# Autodesk Inventor assembly: 4th 5th and 6th Axes Model Assembly
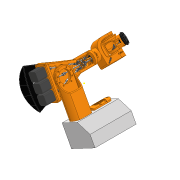
[picture p0: Inventor's stored thumbnail of the model, 180x180]
Saved by Autodesk Inventor 2020 (Build 240168000, 168)
## iProperties
Created: 2021-06-26
Part Number: 4th 5th and 6th Axes Model Assembly
Document SubType Name: Assembly
Designer: Coy
Author: Coy
## Documents named in this file (39)
- E:\Documents\3D Files\Project 3D Models\Industrial 6 Axis Robot Arm\4th 5th amd 6th axis model\4th 5th and 6th Axes Model Assembly.iam
- E:\Documents\3D Files\Project 3D Models\Industrial 6 Axis Robot Arm\4th 5th amd 6th axis model\4th Axis Barrel.ipt
- E:\Documents\3D Files\Project 3D Models\Industrial 6 Axis Robot Arm\4th 5th amd 6th axis model\40mm Bearing.ipt
- E:\Documents\3D Files\Project 3D Models\Industrial 6 Axis Robot Arm\4th 5th amd 6th axis model\5th Axis Tube.ipt
- E:\Documents\3D Files\Project 3D Models\Industrial 6 Axis Robot Arm\4th 5th amd 6th axis model\5x100mm Rod.ipt
- E:\Documents\3D Files\Project 3D Models\Industrial 6 Axis Robot Arm\4th 5th amd 6th axis model\3rd Axis.ipt
- E:\Documents\3D Files\Project 3D Models\Industrial 6 Axis Robot Arm\4th 5th amd 6th axis model\5x8x2.5mm Bearing.ipt
- E:\Documents\3D Files\Project 3D Models\Industrial 6 Axis Robot Arm\4th 5th amd 6th axis model\12x28x8mm Bearing.ipt
- E:\Documents\3D Files\Project 3D Models\Industrial 6 Axis Robot Arm\4th 5th amd 6th axis model\4th Axis Drive Gears.ipt
- E:\Documents\3D Files\Project 3D Models\Industrial 6 Axis Robot Arm\4th 5th amd 6th axis model\6th Axis Drive Gear.ipt
- E:\Documents\3D Files\Project 3D Models\Industrial 6 Axis Robot Arm\4th 5th amd 6th axis model\5x60mm Rod.ipt
- E:\Documents\3D Files\Project 3D Models\Industrial 6 Axis Robot Arm\4th 5th amd 6th axis model\4th Axis Main Drive Gear.ipt
- E:\Documents\3D Files\Project 3D Models\Industrial 6 Axis Robot Arm\4th 5th amd 6th axis model\5th Axis Drive Gear.ipt
- E:\Documents\3D Files\Project 3D Models\Industrial 6 Axis Robot Arm\4th 5th amd 6th axis model\5x42mm Rod.ipt
- E:\Documents\3D Files\Project 3D Models\Industrial 6 Axis Robot Arm\4th 5th amd 6th axis model\5x31mm Rod.ipt
- E:\Documents\3D Files\Project 3D Models\Industrial 6 Axis Robot Arm\4th 5th amd 6th axis model\5x24mm Universal Joint\Assembly.iam
- E:\Documents\3D Files\Project 3D Models\Industrial 6 Axis Robot Arm\4th 5th amd 6th axis model\Nema 17 Stepper Motor.ipt
- E:\Documents\3D Files\Project 3D Models\Industrial 6 Axis Robot Arm\4th 5th amd 6th axis model\5x61.5mm Rod.ipt
- E:\Documents\3D Files\Project 3D Models\Industrial 6 Axis Robot Arm\4th 5th amd 6th axis model\5mm Coupler.ipt
- E:\Documents\3D Files\Project 3D Models\Industrial 6 Axis Robot Arm\4th 5th amd 6th axis model\5x67.3mm Rod.ipt
- E:\Documents\3D Files\Downloaded 3D Files\GrabCad Downloads\gt2-belt-timing-gears-1.snapshot.15\STEP\Gear-5mm-36teeth.ipt
- E:\Documents\3D Files\Downloaded 3D Files\GrabCad Downloads\gt2-belt-timing-gears-1.snapshot.15\STEP\Gear-10mm-36teeth.ipt
- E:\Documents\3D Files\Project 3D Models\Industrial 6 Axis Robot Arm\4th 5th amd 6th axis model\GT2 Idler Pulley.ipt
- E:\Documents\3D Files\Project 3D Models\Industrial 6 Axis Robot Arm\4th 5th amd 6th axis model\M5 60mm Threaded Rod.ipt
- E:\Documents\3D Files\Project 3D Models\Industrial 6 Axis Robot Arm\4th 5th amd 6th axis model\Axis 6 Gearbox.ipt
- E:\Documents\3D Files\Project 3D Models\Industrial 6 Axis Robot Arm\4th 5th amd 6th axis model\Axis 5 Drive Rod.ipt
- E:\Documents\3D Files\Project 3D Models\Industrial 6 Axis Robot Arm\4th 5th amd 6th axis model\Mounting Plate.ipt
- E:\Documents\3D Files\Project 3D Models\Industrial 6 Axis Robot Arm\4th 5th amd 6th axis model\25x37x7mm Bearing.ipt
- E:\Documents\3D Files\Project 3D Models\Industrial 6 Axis Robot Arm\4th 5th amd 6th axis model\5x37.5mm Rod.ipt
- E:\Documents\3D Files\Project 3D Models\Industrial 6 Axis Robot Arm\4th 5th amd 6th axis model\5x45.75mm Rod.ipt
- E:\Documents\3D Files\Project 3D Models\Industrial 6 Axis Robot Arm\4th 5th amd 6th axis model\Corner Gear.ipt
- E:\Documents\3D Files\Project 3D Models\Industrial 6 Axis Robot Arm\4th 5th amd 6th axis model\5th Axis Cover.ipt
- E:\Documents\3D Files\Project 3D Models\Industrial 6 Axis Robot Arm\4th 5th amd 6th axis model\Motor Gard.ipt
- E:\Documents\3D Files\Project 3D Models\Industrial 6 Axis Robot Arm\4th 5th amd 6th axis model\Axis 2 Arm.ipt
- E:\Documents\3D Files\Project 3D Models\Industrial 6 Axis Robot Arm\4th 5th amd 6th axis model\Axis 6 Gearbox Bearing Attchment.ipt
- E:\Documents\3D Files\Project 3D Models\Industrial 6 Axis Robot Arm\4th 5th amd 6th axis model\KR500 0.25 Model Stand.ipt
- E:\Documents\3D Files\Project 3D Models\Industrial 6 Axis Robot Arm\4th 5th amd 6th axis model\3rd Axis Motor Mounts.ipt
- E:\Documents\3D Files\Project 3D Models\Industrial 6 Axis Robot Arm\4th 5th amd 6th axis model\GT2 Idler Pulley No Walls.ipt
- C:\Users\Coy\Downloads\2664N316_METAL GEAR - 20 DEGREE PRESSURE ANGLE.ipt
## Components (80 placed, 38 different names)
1. 4th Axis Barrel:1 — Mate:1, Mate:2, Mate:14, Flush:4, Mate:21, Rotation:2, Rotation:3, Flush:33, Mate:71, Flush:34, Flush:35, Flush:38, Flush:39, Mate:107, Flush:51, Mate:108, Mate:119, Mate:128
2. 40mm Bearing:1 — Mate:1, Mate:2, Mate:10
3. 5th Axis Tube:1 — Flush:1, Flush:2, Mate:13, Mate:16, Flush:3, Flush:4, Flush:21, Flush:22, Rotation:14, Flush:36, Rotation:29
4. 5x100mm Rod:1 — Mate:11, Mate:12, Mate:15, Mate:16, Flush:3, Mate:22, Flush:10, Rotation:4, Mate:27, Flush:37, Rotation:30
5. 3rd Axis:1 — Mate:10, Mate:15, Mate:17, Mate:18, Flush:7, Flush:8, Mate:21, Mate:28, Flush:14, Mate:29, Flush:15, Mate:30, Flush:16, Mate:31, Flush:17, Mate:32, Flush:18, Mate:40, Flush:25, Mate:41, Flush:26, Angle:1, Angle:2, Angle:3, Mate:110, Mate:111, Mate:112, Mate:113, Mate:114, Mate:122, Mate:123, Mate:124
6. 5x8x2.5mm Bearing:1 — Mate:11, Flush:1
7. 5x8x2.5mm Bearing:2 — Mate:12, Flush:2
8. 12x28x8mm Bearing:1 — Mate:13, Mate:14
9. 4th Axis Drive Gears:1 — Mate:20, Rotation:3, Flush:12
10. 4th Axis Drive Gears:2 — Mate:19, Rotation:2, Flush:11
11. 5x8x2.5mm Bearing:3 — Mate:17, Flush:7, Mate:19, Mate:23
12. 5x8x2.5mm Bearing:4 — Mate:18, Flush:8, Mate:20, Mate:24
13. 6th Axis Drive Gear:1 — Mate:22, Flush:10, Rotation:4, Flush:23, Flush:24, Rotation:15
14. 5x60mm Rod:1 — Mate:23, Flush:11, Rotation:10
15. 5x60mm Rod:2 — Mate:24, Flush:12, Mate:34, Rotation:8
16. 5x100mm Rod:2 — Mate:25, Flush:13, Mate:27, Mate:33, Mate:64, Mate:65, Mate:67, Rotation:27
17. 4th Axis Drive Gears:3 — Mate:25, Flush:13, Flush:19, Rotation:9, Flush:20
18. 4th Axis Main Drive Gear:1 — Mate:34, Flush:19, Rotation:8, Rotation:9
19. 4th Axis Main Drive Gear:2 — Flush:20, Rotation:10
20. 5x8x2.5mm Bearing:5 — Mate:28, Flush:14
21. 5x8x2.5mm Bearing:6 — Mate:31, Flush:17, Mate:33
22. 5x8x2.5mm Bearing:7 — Mate:29, Flush:15
23. 5x8x2.5mm Bearing:8 — Mate:32, Flush:18, Mate:36
24. 5x8x2.5mm Bearing:9 — Mate:30, Flush:16, Mate:38
25. 5th Axis Drive Gear:1 — Flush:21, Rotation:13, Mate:37, Rotation:14
26. 5x42mm Rod:1 — Mate:36, Flush:22, Rotation:13, Mate:37, Mate:42, Flush:27, Rotation:17
27. 5x31mm Rod:1 — Mate:38, Flush:23, Mate:39, Rotation:16, Mate:43, Flush:28, Rotation:18
28. 5th Axis Drive Gear:2 — Mate:39, Flush:24, Rotation:15, Rotation:16
29. 5x8x2.5mm Bearing:10 — Mate:40, Flush:25
30. 5x8x2.5mm Bearing:11 — Mate:41, Flush:26
31. Assembly:1 [sub-assembly] — Mate:42, Flush:27, Rotation:17, Mate:57, Rotation:21, Rotation:22
32. Assembly:2 [sub-assembly] — Mate:43, Flush:28, Rotation:18, Mate:62, Rotation:25, Mate:63
33. Nema 17 Stepper Motor:1 — Angle:1, Mate:50, Flush:29
34. Nema 17 Stepper Motor:2 — Angle:2, Mate:68, Mate:69
35. Nema 17 Stepper Motor:3 — Angle:3, Mate:51, Flush:30
36. Assembly:3 [sub-assembly] — Mate:50, Flush:29, Flush:31, Mate:56, Rotation:22
37. Assembly:4 [sub-assembly] — Mate:51, Flush:30, Mate:62, Rotation:25, Flush:32
38. 5x61.5mm Rod:1 — Mate:58, Mate:59, Mate:61, Rotation:23, Rotation:24, Flush:32
39. 5x61.5mm Rod:2 — Mate:60, Mate:61, Rotation:24, Mate:63
40. 5x61.5mm Rod:3 — Mate:52, Mate:53, Mate:55, Rotation:19, Rotation:20, Flush:31, Mate:56
41. 5x61.5mm Rod:4 — Mate:54, Mate:55, Rotation:20, Mate:57, Rotation:21
42. 5mm Coupler:1 — Mate:58, Mate:59, Mate:60, Rotation:23
43. 5mm Coupler:2 — Mate:52, Mate:53, Mate:54, Rotation:19
44. 5x67.3mm Rod:1 — Mate:66, Mate:67, Rotation:27, Rotation:28
45. 5mm Coupler:3 — Mate:64, Mate:65, Mate:66
46. 5mm Coupler:4 — Mate:68, Mate:69, Rotation:28
47. 12x28x8mm Bearing:2 — Flush:33
48. 12x28x8mm Bearing:3 — Mate:71, Flush:34, Mate:118
49. 12x28x8mm Bearing:4 — Flush:35, Mate:76, Mate:77, Mate:86
50. Gear-5mm-36teeth:1 — Flush:37, Rotation:30, Rotation:34
51. Gear-10mm-36teeth:1 — Flush:36, Rotation:29, Rotation:36
52. GT2 Idler Pulley:1 — Mate:82, Flush:54
53. Gear-10mm-36teeth:2 — Mate:76, Mate:77, Mate:78, Mate:79, Flush:48, Rotation:34, Rotation:41
54. Gear-5mm-36teeth:2 — Mate:78, Mate:79, Rotation:35, Rotation:36
55. M5 60mm Threaded Rod:1 — Flush:38, Mate:82, Mate:88
56. M5 60mm Threaded Rod:2 — Flush:39, Mate:126, Mate:127, Mate:128
57. Axis 6 Gearbox:1 — Flush:40, Rotation:31, Flush:44, Mate:93, Flush:45, Mate:95, Mate:101, Flush:46, Mate:102, Flush:47, Mate:115, Mate:116, Mate:117, Rotation:41
58. Axis 5 Drive Rod:1 — Mate:86, Flush:40, Rotation:31, Mate:91, Flush:43, Mate:92
59. GT2 Idler Pulley:3 — Mate:88, Flush:55
60. 5x8x2.5mm Bearing:12 — Mate:91, Flush:43
61. 5x8x2.5mm Bearing:13 — Mate:92, Flush:44, Mate:104
62. Mounting Plate:1 — Mate:94, Mate:95, Mate:99, Rotation:40
63. 25x37x7mm Bearing:1 — Mate:93, Flush:45, Mate:94
64. 5x8x2.5mm Bearing:14 — Mate:98, Mate:101, Flush:46
65. 5x8x2.5mm Bearing:15 — Mate:102, Flush:47, Mate:103
66. 5x37.5mm Rod:1 — Mate:98, Mate:99, Mate:100, Rotation:32, Mate:105, Rotation:38, Flush:50
67. 4th Axis Drive Gears:4 — Mate:100, Rotation:32, Mate:103, Rotation:40
68. 5x45.75mm Rod:1 — Mate:104, Flush:48, Rotation:35, Mate:106, Flush:49, Rotation:37
69. Corner Gear:1 — Mate:105, Rotation:38, Rotation:39, Flush:50
70. Corner Gear:2 — Mate:106, Flush:49, Rotation:37, Rotation:39
71. 5th Axis Cover:1 — Mate:107, Flush:51, Mate:108
72. Motor Gard:1 — Mate:110, Mate:111
73. Axis 2 Arm:1 — Mate:112, Mate:113, Mate:114, Mate:120, Flush:52, Flush:53
74. Axis 6 Gearbox Bearing Attchment:1 — Mate:115, Mate:116, Mate:117, Mate:118, Mate:119
75. KR500 0.25 Model Stand:1 — Mate:120, Flush:52, Flush:53, Mate:121
76. 5th Axis Cover:2 — Mate:121
77. 3rd Axis Motor Mounts:1 — Mate:122, Mate:123, Mate:124
78. GT2 Idler Pulley No Walls:1 — Mate:126, Flush:55
79. GT2 Idler Pulley No Walls:2 — Mate:127, Flush:54
80. 2664N316_METAL GEAR - 20 DEGREE PRESSURE ANGLE:1
## Relationships (182: Mate 96, Flush 50, RelateRotation 33, Angle 3)
- Mate:1: 4th Axis Barrel:1 ↔ 40mm Bearing:1
- Mate:2 (0.2 mm): 4th Axis Barrel:1 ↔ 40mm Bearing:1
- Mate:10 (0.2 mm): 40mm Bearing:1 ↔ 3rd Axis:1
- Mate:11: 5x100mm Rod:1 ↔ 5x8x2.5mm Bearing:1
- Mate:12: 5x100mm Rod:1 ↔ 5x8x2.5mm Bearing:2
- Flush:1: 5th Axis Tube:1 ↔ 5x8x2.5mm Bearing:1
- Flush:2: 5th Axis Tube:1 ↔ 5x8x2.5mm Bearing:2
- Mate:13: 5th Axis Tube:1 ↔ 12x28x8mm Bearing:1
- Mate:14 (0.2 mm): 4th Axis Barrel:1 ↔ 12x28x8mm Bearing:1
- Mate:15: 5x100mm Rod:1 ↔ 3rd Axis:1
- Mate:16: 5th Axis Tube:1 ↔ 5x100mm Rod:1
- Flush:3 (11 mm): 5th Axis Tube:1 ↔ 5x100mm Rod:1
- Flush:4 (-26 mm): 4th Axis Barrel:1 ↔ 5th Axis Tube:1
- Mate:17: 3rd Axis:1 ↔ 5x8x2.5mm Bearing:3
- Mate:18: 3rd Axis:1 ↔ 5x8x2.5mm Bearing:4
- Flush:7: 3rd Axis:1 ↔ 5x8x2.5mm Bearing:3
- Flush:8: 3rd Axis:1 ↔ 5x8x2.5mm Bearing:4
- Mate:19: 4th Axis Drive Gears:2 ↔ 5x8x2.5mm Bearing:3
- Mate:20: 4th Axis Drive Gears:1 ↔ 5x8x2.5mm Bearing:4
- Mate:21: 4th Axis Barrel:1 ↔ 3rd Axis:1
- Rotation:2 [RelateRotation] (0.2917 ul): 4th Axis Barrel:1 ↔ 4th Axis Drive Gears:2
- Rotation:3 [RelateRotation] (0.2917 ul): 4th Axis Barrel:1 ↔ 4th Axis Drive Gears:1
- Mate:22: 5x100mm Rod:1 ↔ 6th Axis Drive Gear:1
- Flush:10: 5x100mm Rod:1 ↔ 6th Axis Drive Gear:1
- Rotation:4 [RelateRotation] (1 ul): 5x100mm Rod:1 ↔ 6th Axis Drive Gear:1
- Mate:23: 5x8x2.5mm Bearing:3 ↔ 5x60mm Rod:1
- Flush:11: 4th Axis Drive Gears:2 ↔ 5x60mm Rod:1
- Mate:24: 5x8x2.5mm Bearing:4 ↔ 5x60mm Rod:2
- Flush:12: 4th Axis Drive Gears:1 ↔ 5x60mm Rod:2
- Mate:25: 5x100mm Rod:2 ↔ 4th Axis Drive Gears:3
- Flush:13: 5x100mm Rod:2 ↔ 4th Axis Drive Gears:3
- Mate:27 (5 mm): 5x100mm Rod:1 ↔ 5x100mm Rod:2
- Mate:28: 3rd Axis:1 ↔ 5x8x2.5mm Bearing:5
- Flush:14: 3rd Axis:1 ↔ 5x8x2.5mm Bearing:5
- Mate:29: 3rd Axis:1 ↔ 5x8x2.5mm Bearing:7
- Flush:15: 3rd Axis:1 ↔ 5x8x2.5mm Bearing:7
- Mate:30: 3rd Axis:1 ↔ 5x8x2.5mm Bearing:9
- Flush:16: 3rd Axis:1 ↔ 5x8x2.5mm Bearing:9
- Mate:31: 3rd Axis:1 ↔ 5x8x2.5mm Bearing:6
- Flush:17: 3rd Axis:1 ↔ 5x8x2.5mm Bearing:6
- Mate:32: 3rd Axis:1 ↔ 5x8x2.5mm Bearing:8
- Flush:18: 3rd Axis:1 ↔ 5x8x2.5mm Bearing:8
- Mate:33: 5x100mm Rod:2 ↔ 5x8x2.5mm Bearing:6
- Mate:34: 5x60mm Rod:2 ↔ 4th Axis Main Drive Gear:1
- Flush:19: 4th Axis Drive Gears:3 ↔ 4th Axis Main Drive Gear:1
- Rotation:8 [RelateRotation] (1 ul): 5x60mm Rod:2 ↔ 4th Axis Main Drive Gear:1
- Rotation:9 [RelateRotation] (1.4286 ul): 4th Axis Drive Gears:3 ↔ 4th Axis Main Drive Gear:1
- Flush:20: 4th Axis Drive Gears:3 ↔ 4th Axis Main Drive Gear:2
- Rotation:10 [RelateRotation] (1 ul): 5x60mm Rod:1 ↔ 4th Axis Main Drive Gear:2
- Flush:21: 5th Axis Tube:1 ↔ 5th Axis Drive Gear:1
- Mate:36: 5x8x2.5mm Bearing:8 ↔ 5x42mm Rod:1
- Flush:22: 5th Axis Tube:1 ↔ 5x42mm Rod:1
- Rotation:13 [RelateRotation] (1 ul): 5th Axis Drive Gear:1 ↔ 5x42mm Rod:1
- Mate:37: 5th Axis Drive Gear:1 ↔ 5x42mm Rod:1
- Rotation:14 [RelateRotation] (0.5 ul): 5th Axis Tube:1 ↔ 5th Axis Drive Gear:1
- Mate:38: 5x8x2.5mm Bearing:9 ↔ 5x31mm Rod:1
- Flush:23: 6th Axis Drive Gear:1 ↔ 5x31mm Rod:1
- Mate:39: 5x31mm Rod:1 ↔ 5th Axis Drive Gear:2
- Flush:24: 6th Axis Drive Gear:1 ↔ 5th Axis Drive Gear:2
- Rotation:15 [RelateRotation] (0.5 ul): 6th Axis Drive Gear:1 ↔ 5th Axis Drive Gear:2
- Rotation:16 [RelateRotation] (1 ul): 5x31mm Rod:1 ↔ 5th Axis Drive Gear:2
- Mate:40: 3rd Axis:1 ↔ 5x8x2.5mm Bearing:10
- Flush:25: 3rd Axis:1 ↔ 5x8x2.5mm Bearing:10
- Mate:41: 3rd Axis:1 ↔ 5x8x2.5mm Bearing:11
- Flush:26: 3rd Axis:1 ↔ 5x8x2.5mm Bearing:11
- Mate:42: 5x42mm Rod:1 ↔ Assembly:1
- Flush:27: 5x42mm Rod:1 ↔ Assembly:1
- Mate:43: 5x31mm Rod:1 ↔ Assembly:2
- Flush:28: 5x31mm Rod:1 ↔ Assembly:2
- Rotation:17 [RelateRotation] (1 ul): 5x42mm Rod:1 ↔ Assembly:1
- Rotation:18 [RelateRotation] (1 ul): 5x31mm Rod:1 ↔ Assembly:2
- Angle:1 (0 deg): 3rd Axis:1 ↔ Nema 17 Stepper Motor:1
- Angle:2 (0 deg): 3rd Axis:1 ↔ Nema 17 Stepper Motor:2
- Angle:3 (0 deg): 3rd Axis:1 ↔ Nema 17 Stepper Motor:3
- Mate:50: Nema 17 Stepper Motor:1 ↔ Assembly:3
- Flush:29: Nema 17 Stepper Motor:1 ↔ Assembly:3
- Mate:51: Nema 17 Stepper Motor:3 ↔ Assembly:4
- Flush:30: Nema 17 Stepper Motor:3 ↔ Assembly:4
- Mate:52: 5x61.5mm Rod:3 ↔ 5mm Coupler:2
- Mate:53 (-6 mm): 5x61.5mm Rod:3 ↔ 5mm Coupler:2
- Mate:54: 5x61.5mm Rod:4 ↔ 5mm Coupler:2
- Mate:55: 5x61.5mm Rod:3 ↔ 5x61.5mm Rod:4
- Rotation:19 [RelateRotation] (1 ul): 5x61.5mm Rod:3 ↔ 5mm Coupler:2
- Rotation:20 [RelateRotation] (1 ul): 5x61.5mm Rod:3 ↔ 5x61.5mm Rod:4
- Flush:31: Assembly:3 ↔ 5x61.5mm Rod:3
- Mate:56: Assembly:3 ↔ 5x61.5mm Rod:3
- Mate:57: Assembly:1 ↔ 5x61.5mm Rod:4
- Rotation:21 [RelateRotation] (1 ul): Assembly:1 ↔ 5x61.5mm Rod:4
- Rotation:22 [RelateRotation] (1 ul): Assembly:1 ↔ Assembly:3
- Mate:58: 5x61.5mm Rod:1 ↔ 5mm Coupler:1
- Mate:59 (-6 mm): 5x61.5mm Rod:1 ↔ 5mm Coupler:1
- Mate:60: 5x61.5mm Rod:2 ↔ 5mm Coupler:1
- Mate:61: 5x61.5mm Rod:1 ↔ 5x61.5mm Rod:2
- Rotation:23 [RelateRotation] (1 ul): 5x61.5mm Rod:1 ↔ 5mm Coupler:1
- Rotation:24 [RelateRotation] (1 ul): 5x61.5mm Rod:1 ↔ 5x61.5mm Rod:2
- Mate:62: Assembly:2 ↔ Assembly:4
- Rotation:25 [RelateRotation] (1 ul): Assembly:2 ↔ Assembly:4
- Flush:32: Assembly:4 ↔ 5x61.5mm Rod:1
- Mate:63: Assembly:2 ↔ 5x61.5mm Rod:2
- Mate:64: 5x100mm Rod:2 ↔ 5mm Coupler:3
- Mate:65 (-6 mm): 5x100mm Rod:2 ↔ 5mm Coupler:3
- Mate:66: 5x67.3mm Rod:1 ↔ 5mm Coupler:3
- Mate:67: 5x100mm Rod:2 ↔ 5x67.3mm Rod:1
- Mate:68: Nema 17 Stepper Motor:2 ↔ 5mm Coupler:4
- Mate:69 (-6 mm): Nema 17 Stepper Motor:2 ↔ 5mm Coupler:4
- Rotation:27 [RelateRotation] (1 ul): 5x100mm Rod:2 ↔ 5x67.3mm Rod:1
- Rotation:28 [RelateRotation] (1 ul): 5x67.3mm Rod:1 ↔ 5mm Coupler:4
- Flush:33: 4th Axis Barrel:1 ↔ 12x28x8mm Bearing:2
- Mate:71: 4th Axis Barrel:1 ↔ 12x28x8mm Bearing:3
- Flush:34: 4th Axis Barrel:1 ↔ 12x28x8mm Bearing:3
- Flush:35: 4th Axis Barrel:1 ↔ 12x28x8mm Bearing:4
- Flush:36: 5th Axis Tube:1 ↔ Gear-10mm-36teeth:1
- Rotation:29 [RelateRotation] (1 ul): 5th Axis Tube:1 ↔ Gear-10mm-36teeth:1
- Flush:37: 5x100mm Rod:1 ↔ Gear-5mm-36teeth:1
- Rotation:30 [RelateRotation] (1 ul): 5x100mm Rod:1 ↔ Gear-5mm-36teeth:1
- Mate:76: 12x28x8mm Bearing:4 ↔ Gear-10mm-36teeth:2
- Mate:77 (0.5 mm): 12x28x8mm Bearing:4 ↔ Gear-10mm-36teeth:2
- Mate:78: Gear-10mm-36teeth:2 ↔ Gear-5mm-36teeth:2
- Mate:79 (0.5 mm): Gear-10mm-36teeth:2 ↔ Gear-5mm-36teeth:2
- Flush:38 (-4 mm): 4th Axis Barrel:1 ↔ M5 60mm Threaded Rod:1
- Flush:39 (-4 mm): 4th Axis Barrel:1 ↔ M5 60mm Threaded Rod:2
- Mate:82: GT2 Idler Pulley:1 ↔ M5 60mm Threaded Rod:1
- Mate:86: 12x28x8mm Bearing:4 ↔ Axis 5 Drive Rod:1
- Flush:40: Axis 6 Gearbox:1 ↔ Axis 5 Drive Rod:1
- Rotation:31 [RelateRotation] (1 ul): Axis 6 Gearbox:1 ↔ Axis 5 Drive Rod:1
- Mate:88: M5 60mm Threaded Rod:1 ↔ GT2 Idler Pulley:3
- Mate:91: Axis 5 Drive Rod:1 ↔ 5x8x2.5mm Bearing:12
- Flush:43: Axis 5 Drive Rod:1 ↔ 5x8x2.5mm Bearing:12
- Mate:92: Axis 5 Drive Rod:1 ↔ 5x8x2.5mm Bearing:13
- Flush:44: Axis 6 Gearbox:1 ↔ 5x8x2.5mm Bearing:13
- Mate:93: Axis 6 Gearbox:1 ↔ 25x37x7mm Bearing:1
- Flush:45: Axis 6 Gearbox:1 ↔ 25x37x7mm Bearing:1
- Mate:94: Mounting Plate:1 ↔ 25x37x7mm Bearing:1
- Mate:95: Axis 6 Gearbox:1 ↔ Mounting Plate:1
- Mate:98: 5x8x2.5mm Bearing:14 ↔ 5x37.5mm Rod:1
- Mate:99 (0.5 mm): Mounting Plate:1 ↔ 5x37.5mm Rod:1
- Mate:100: 5x37.5mm Rod:1 ↔ 4th Axis Drive Gears:4
- Rotation:32 [RelateRotation] (1 ul): 5x37.5mm Rod:1 ↔ 4th Axis Drive Gears:4
- Mate:101: Axis 6 Gearbox:1 ↔ 5x8x2.5mm Bearing:14
- Flush:46: Axis 6 Gearbox:1 ↔ 5x8x2.5mm Bearing:14
- Mate:102: Axis 6 Gearbox:1 ↔ 5x8x2.5mm Bearing:15
- Flush:47: Axis 6 Gearbox:1 ↔ 5x8x2.5mm Bearing:15
- Mate:103 (0.2 mm): 5x8x2.5mm Bearing:15 ↔ 4th Axis Drive Gears:4
- Mate:104: 5x8x2.5mm Bearing:13 ↔ 5x45.75mm Rod:1
- Flush:48 (-10 mm): Gear-10mm-36teeth:2 ↔ 5x45.75mm Rod:1
- Rotation:34 [RelateRotation] (1 ul): Gear-5mm-36teeth:1 ↔ Gear-10mm-36teeth:2
- Rotation:35 [RelateRotation] (1 ul): Gear-5mm-36teeth:2 ↔ 5x45.75mm Rod:1
- Rotation:36 [RelateRotation] (1 ul): Gear-10mm-36teeth:1 ↔ Gear-5mm-36teeth:2
- Mate:105: 5x37.5mm Rod:1 ↔ Corner Gear:1
- Mate:106: 5x45.75mm Rod:1 ↔ Corner Gear:2
- Flush:49 (2 mm): 5x45.75mm Rod:1 ↔ Corner Gear:2
- Rotation:37 [RelateRotation] (1 ul): 5x45.75mm Rod:1 ↔ Corner Gear:2
- Rotation:38 [RelateRotation] (1 ul): 5x37.5mm Rod:1 ↔ Corner Gear:1
- Rotation:39 [RelateRotation] (1 ul): Corner Gear:1 ↔ Corner Gear:2
- Rotation:40 [RelateRotation] (0.4667 ul): Mounting Plate:1 ↔ 4th Axis Drive Gears:4
- Flush:50 (3.3 mm): 5x37.5mm Rod:1 ↔ Corner Gear:1
- Mate:107: 4th Axis Barrel:1 ↔ 5th Axis Cover:1
- Flush:51: 4th Axis Barrel:1 ↔ 5th Axis Cover:1
- Mate:108: 4th Axis Barrel:1 ↔ 5th Axis Cover:1
- Mate:110: 3rd Axis:1 ↔ Motor Gard:1
- Mate:111: 3rd Axis:1 ↔ Motor Gard:1
- Mate:112: 3rd Axis:1 ↔ Axis 2 Arm:1
- Mate:113: 3rd Axis:1 ↔ Axis 2 Arm:1
- Mate:114: 3rd Axis:1 ↔ Axis 2 Arm:1
- Mate:115: Axis 6 Gearbox:1 ↔ Axis 6 Gearbox Bearing Attchment:1
- Mate:116: Axis 6 Gearbox:1 ↔ Axis 6 Gearbox Bearing Attchment:1
- Mate:117 (0.5 mm): Axis 6 Gearbox:1 ↔ Axis 6 Gearbox Bearing Attchment:1
- Mate:118: 12x28x8mm Bearing:3 ↔ Axis 6 Gearbox Bearing Attchment:1
- Mate:119 (0.25 mm): 4th Axis Barrel:1 ↔ Axis 6 Gearbox Bearing Attchment:1
- Rotation:41 [RelateRotation] (1 ul): Gear-10mm-36teeth:2 ↔ Axis 6 Gearbox:1
- Mate:120: Axis 2 Arm:1 ↔ KR500 0.25 Model Stand:1
- Flush:52 (10 mm): Axis 2 Arm:1 ↔ KR500 0.25 Model Stand:1
- Flush:53 (35 mm): Axis 2 Arm:1 ↔ KR500 0.25 Model Stand:1
- Mate:121: KR500 0.25 Model Stand:1 ↔ 5th Axis Cover:2
- Mate:122 (0.5 mm): 3rd Axis:1 ↔ 3rd Axis Motor Mounts:1
- Mate:123: 3rd Axis:1 ↔ 3rd Axis Motor Mounts:1
- Mate:124: 3rd Axis:1 ↔ 3rd Axis Motor Mounts:1
- Mate:126: M5 60mm Threaded Rod:2 ↔ GT2 Idler Pulley No Walls:1
- Mate:127: M5 60mm Threaded Rod:2 ↔ GT2 Idler Pulley No Walls:2
- Flush:54: GT2 Idler Pulley:1 ↔ GT2 Idler Pulley No Walls:2
- Flush:55: GT2 Idler Pulley:3 ↔ GT2 Idler Pulley No Walls:1
- Mate:128: 4th Axis Barrel:1 ↔ M5 60mm Threaded Rod:2
